# Autodesk Inventor assembly: MTM_itemFrame
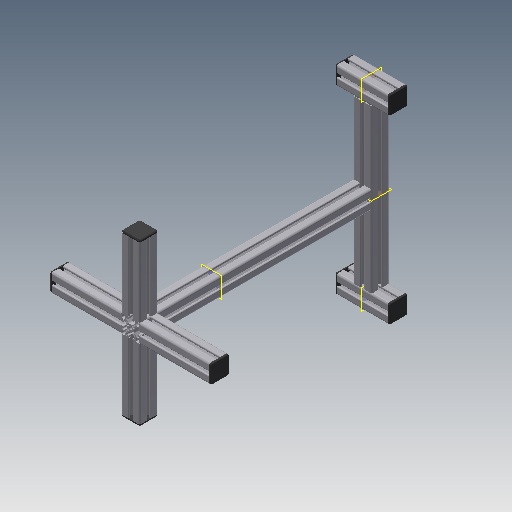
[picture p0: Inventor's stored thumbnail of the model, 512x512]
Saved by Autodesk Inventor 2021.4 (Build 254397000, 397)
## iProperties
Created: 2022-08-02
Part Number: MTM_itemFrame
Material: Generisch
Document SubType Name: Assembly
Designer: alexw
Mass: 913.316 g
Surface Area: 10074.2 cm^2
Volume: 913.316 cm^3
Density: 1 g/cm^3
Author: alexw
## Documents named in this file (6)
- C:\Users\alexw\Documents\Inventor\Projects\03_CurrentProjects\MasterThesis\TrainingConsol_220422\Workgroups\Workgroup\MTM_itemFrame.iam
- C:\Users\alexw\Documents\Inventor\Projects\03_CurrentProjects\MasterThesis\TrainingConsol_220422\Workgroups\Workgroup\item_7000009_Profile_8_40x40_E_L=110.ipt
- C:\Users\alexw\Documents\Inventor\Projects\03_CurrentProjects\MasterThesis\TrainingConsol_220422\Workgroups\Workgroup\item_7000009_Profile_8_40x40_E_L=350.ipt
- C:\Users\alexw\Documents\Inventor\Projects\03_CurrentProjects\MasterThesis\TrainingConsol_220422\Workgroups\Workgroup\item_0002601_Cap_8_40x40.ipt
- C:\Users\alexw\Documents\Inventor\Projects\03_CurrentProjects\MasterThesis\TrainingConsol_220422\Workgroups\Workgroup\item_7000009_Profile_8_40x40_E_L=150.ipt
- C:\Users\alexw\Documents\Inventor\Projects\03_CurrentProjects\MasterThesis\TrainingConsol_220422\Workgroups\Workgroup\ItemFrame_TopQuerstrebe.ipt
## Components (16 placed, 5 different names)
1. item_7000009_Profile_8_40x40_E_L=110:1 — Flush:29, Mate:15, Mate:16, Flush:31, Mate:17, Mate:18, Mate:26
2. item_7000009_Profile_8_40x40_E_L=110:2 — Mate:19, Flush:32, Mate:20, Mate:21, Mate:22, Mate:23, Mate:24
3. ItemFrame_TopQuerstrebe:1 — Flush:29, Flush:30, Flush:31, Mate:19, Flush:32, Mate:20, Mate:25, Mate:26
4. item_7000009_Profile_8_40x40_E_L=350:2 — Flush:26, Flush:27, Flush:28, Flush:30, Mate:25
5. item_0002601_Cap_8_40x40:1 — Mate:15, Mate:16
6. item_0002601_Cap_8_40x40:2 — Mate:21, Mate:22
7. item_7000009_Profile_8_40x40_E_L=150:1
8. item_7000009_Profile_8_40x40_E_L=150:2
9. item_7000009_Profile_8_40x40_E_L=150:3
10. item_7000009_Profile_8_40x40_E_L=150:4
11. item_0002601_Cap_8_40x40:3
12. item_0002601_Cap_8_40x40:4
13. item_0002601_Cap_8_40x40:5
14. item_0002601_Cap_8_40x40:6
15. item_0002601_Cap_8_40x40:7 — Mate:17, Mate:18
16. item_0002601_Cap_8_40x40:8 — Mate:23, Mate:24
## Relationships (44: Flush 24, Mate 20)
- [Flush]: ItemFrame_TopQuerstrebe:1 ↔ item_7000009_Profile_8_40x40_E_L=350:2
- [Flush]: item_7000009_Profile_8_40x40_E_L=350:2 ↔ item_7000009_Profile_8_40x40_E_L=150:2
- [Flush]: item_7000009_Profile_8_40x40_E_L=350:2 ↔ item_7000009_Profile_8_40x40_E_L=150:4
- [Flush]: item_7000009_Profile_8_40x40_E_L=350:2 ↔ item_7000009_Profile_8_40x40_E_L=150:4
- [Flush]: item_7000009_Profile_8_40x40_E_L=350:2 ↔ item_7000009_Profile_8_40x40_E_L=150:2
- [Mate]: item_7000009_Profile_8_40x40_E_L=350:2 ↔ item_7000009_Profile_8_40x40_E_L=150:4
- [Mate]: item_7000009_Profile_8_40x40_E_L=350:2 ↔ item_7000009_Profile_8_40x40_E_L=150:3
- [Mate]: item_7000009_Profile_8_40x40_E_L=350:2 ↔ item_7000009_Profile_8_40x40_E_L=150:1
- [Mate]: item_7000009_Profile_8_40x40_E_L=350:2 ↔ item_7000009_Profile_8_40x40_E_L=150:2
- [Flush]: item_7000009_Profile_8_40x40_E_L=350:2 ↔ item_7000009_Profile_8_40x40_E_L=150:3
- [Flush]: item_7000009_Profile_8_40x40_E_L=350:2 ↔ item_7000009_Profile_8_40x40_E_L=150:3
- [Flush]: item_7000009_Profile_8_40x40_E_L=350:2 ↔ item_7000009_Profile_8_40x40_E_L=150:1
- [Flush]: item_7000009_Profile_8_40x40_E_L=350:2 ↔ item_7000009_Profile_8_40x40_E_L=150:1
- [Flush]: item_7000009_Profile_8_40x40_E_L=150:4 ↔ item_0002601_Cap_8_40x40:4
- [Mate]: item_7000009_Profile_8_40x40_E_L=150:4 ↔ item_0002601_Cap_8_40x40:4
- [Mate]: item_7000009_Profile_8_40x40_E_L=150:2 ↔ item_0002601_Cap_8_40x40:3
- [Mate]: item_7000009_Profile_8_40x40_E_L=150:1 ↔ item_0002601_Cap_8_40x40:5
- [Mate]: item_7000009_Profile_8_40x40_E_L=150:3 ↔ item_0002601_Cap_8_40x40:6
- [Flush]: item_7000009_Profile_8_40x40_E_L=150:3 ↔ item_0002601_Cap_8_40x40:6
- [Flush]: item_7000009_Profile_8_40x40_E_L=150:3 ↔ item_0002601_Cap_8_40x40:6
- [Flush]: item_7000009_Profile_8_40x40_E_L=150:2 ↔ item_0002601_Cap_8_40x40:3
- [Flush]: item_7000009_Profile_8_40x40_E_L=150:2 ↔ item_0002601_Cap_8_40x40:3
- [Flush]: item_7000009_Profile_8_40x40_E_L=150:1 ↔ item_0002601_Cap_8_40x40:5
- [Flush]: item_7000009_Profile_8_40x40_E_L=150:1 ↔ item_0002601_Cap_8_40x40:5
- [Flush]: item_7000009_Profile_8_40x40_E_L=150:4 ↔ item_0002601_Cap_8_40x40:4
- Flush:26: item_7000009_Profile_8_40x40_E_L=350:2
- Flush:27: item_7000009_Profile_8_40x40_E_L=350:2
- Flush:28: item_7000009_Profile_8_40x40_E_L=350:2
- Flush:29: item_7000009_Profile_8_40x40_E_L=110:1 ↔ ItemFrame_TopQuerstrebe:1
- Mate:15: item_7000009_Profile_8_40x40_E_L=110:1 ↔ item_0002601_Cap_8_40x40:1
- Mate:16: item_7000009_Profile_8_40x40_E_L=110:1 ↔ item_0002601_Cap_8_40x40:1
- Flush:30: ItemFrame_TopQuerstrebe:1 ↔ item_7000009_Profile_8_40x40_E_L=350:2
- Flush:31: item_7000009_Profile_8_40x40_E_L=110:1 ↔ ItemFrame_TopQuerstrebe:1
- Mate:17: item_7000009_Profile_8_40x40_E_L=110:1 ↔ item_0002601_Cap_8_40x40:7
- Mate:18: item_7000009_Profile_8_40x40_E_L=110:1 ↔ item_0002601_Cap_8_40x40:7
- Mate:19: item_7000009_Profile_8_40x40_E_L=110:2 ↔ ItemFrame_TopQuerstrebe:1
- Flush:32: item_7000009_Profile_8_40x40_E_L=110:2 ↔ ItemFrame_TopQuerstrebe:1
- Mate:20: item_7000009_Profile_8_40x40_E_L=110:2 ↔ ItemFrame_TopQuerstrebe:1
- Mate:21: item_7000009_Profile_8_40x40_E_L=110:2 ↔ item_0002601_Cap_8_40x40:2
- Mate:22: item_7000009_Profile_8_40x40_E_L=110:2 ↔ item_0002601_Cap_8_40x40:2
- Mate:23: item_7000009_Profile_8_40x40_E_L=110:2 ↔ item_0002601_Cap_8_40x40:8
- Mate:24: item_7000009_Profile_8_40x40_E_L=110:2 ↔ item_0002601_Cap_8_40x40:8
- Mate:25: ItemFrame_TopQuerstrebe:1 ↔ item_7000009_Profile_8_40x40_E_L=350:2
- Mate:26: item_7000009_Profile_8_40x40_E_L=110:1 ↔ ItemFrame_TopQuerstrebe:1
